# Autodesk Inventor assembly: Ensamble General
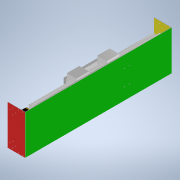
[picture p0: Inventor's stored thumbnail of the model, 180x180]
Saved by Autodesk Inventor 2021 (Build 250183000, 183)
## iProperties
Created: 2022-01-21
Part Number: Ensamble General
Document SubType Name: Assembly
Designer: deuts
Author: deuts
## Documents named in this file (11)
- C:\Users\deuts\Desktop\3dDesigne\SoladuraSemiAutomatizada\Ensamble General.iam
- C:\Users\deuts\Desktop\3dDesigne\SoladuraSemiAutomatizada\Soporte Tuerca.ipt
- C:\Users\deuts\Desktop\3dDesigne\SoladuraSemiAutomatizada\Tornillo 350.ipt
- C:\Users\deuts\Desktop\3dDesigne\SoladuraSemiAutomatizada\Tuerca 16.ipt
- C:\Users\deuts\Desktop\3dDesigne\SoladuraSemiAutomatizada\Acople Flexible.ipt
- C:\Users\deuts\Desktop\3dDesigne\SoladuraSemiAutomatizada\Motor Nema23.ipt
- C:\Users\deuts\Desktop\3dDesigne\SoladuraSemiAutomatizada\Rodamiento lineal.ipt
- C:\Users\deuts\Desktop\3dDesigne\SoladuraSemiAutomatizada\Soporte Motor.ipt
- C:\Users\deuts\Desktop\3dDesigne\SoladuraSemiAutomatizada\Riel.ipt
- C:\Users\deuts\Desktop\3dDesigne\SoladuraSemiAutomatizada\Caja - Base.ipt
- C:\Users\deuts\Desktop\3dDesigne\SoladuraSemiAutomatizada\CajaAux.ipt
## Components (14 placed, 10 different names)
1. Soporte Tuerca:1 — Mate:3, Mate:4, Mate:5, Angle:2, Angle:3, Mate:41, Flush:1, Mate:43, Flush:2
2. Tornillo 350:1 — Mate:3, Mate:6, Mate:7, Angle:1
3. Tuerca 16:1 — Mate:4, Mate:5, Angle:2
4. Acople Flexible:1 — Mate:6, Mate:7, Mate:8, Mate:9, Angle:1
5. Motor Nema23:1 — Mate:8, Mate:9, Angle:3, Mate:38, Angle:6, Mate:39, Flush:3, Flush:4
6. Soporte Motor:1 — Mate:38, Angle:6, Mate:39, Angle:7, Angle:8, Mate:46, Mate:47
7. Rodamiento lineal:1 — Mate:41, Flush:1, Mate:44, Mate:52
8. Rodamiento lineal:2 — Mate:43, Flush:2, Mate:45
9. Riel:1 — Mate:44, Angle:7, Flush:3, Mate:49, Mate:50
10. Riel:2 — Mate:45, Angle:8, Flush:4, Flush:5, Mate:48, Mate:51
11. Caja - Base:1 — Mate:46, Mate:47, Flush:5, Mate:50, Mate:51
12. Rodamiento lineal:3 — Mate:48
13. Rodamiento lineal:4 — Mate:49
14. CajaAux:1 — Mate:52
## Relationships (31: Mate 20, Angle 6, Flush 5)
- Mate:3: Soporte Tuerca:1 ↔ Tornillo 350:1
- Mate:4: Soporte Tuerca:1 ↔ Tuerca 16:1
- Mate:5: Soporte Tuerca:1 ↔ Tuerca 16:1
- Mate:6: Tornillo 350:1 ↔ Acople Flexible:1
- Mate:7 (-12 mm): Tornillo 350:1 ↔ Acople Flexible:1
- Mate:8: Acople Flexible:1 ↔ Motor Nema23:1
- Mate:9 (15 mm): Acople Flexible:1 ↔ Motor Nema23:1
- Angle:1 (0 deg): Tornillo 350:1 ↔ Acople Flexible:1
- Angle:2 (0 deg): Soporte Tuerca:1 ↔ Tuerca 16:1
- Angle:3 (0 deg): Soporte Tuerca:1 ↔ Motor Nema23:1
- Mate:38: Motor Nema23:1 ↔ Soporte Motor:1
- Angle:6 (0 deg): Motor Nema23:1 ↔ Soporte Motor:1
- Mate:39: Motor Nema23:1 ↔ Soporte Motor:1
- Mate:41 (7 mm): Soporte Tuerca:1 ↔ Rodamiento lineal:1
- Flush:1: Soporte Tuerca:1 ↔ Rodamiento lineal:1
- Mate:43 (7 mm): Soporte Tuerca:1 ↔ Rodamiento lineal:2
- Flush:2: Soporte Tuerca:1 ↔ Rodamiento lineal:2
- Mate:44: Rodamiento lineal:1 ↔ Riel:1
- Mate:45: Rodamiento lineal:2 ↔ Riel:2
- Angle:7 (0 deg): Soporte Motor:1 ↔ Riel:1
- Angle:8 (0 deg): Soporte Motor:1 ↔ Riel:2
- Flush:3 (41.7 mm): Motor Nema23:1 ↔ Riel:1
- Flush:4 (41.7 mm): Motor Nema23:1 ↔ Riel:2
- Mate:46: Soporte Motor:1 ↔ Caja - Base:1
- Mate:47: Soporte Motor:1 ↔ Caja - Base:1
- Flush:5 (0.5 mm): Riel:2 ↔ Caja - Base:1
- Mate:48: Riel:2 ↔ Rodamiento lineal:3
- Mate:49: Riel:1 ↔ Rodamiento lineal:4
- Mate:50: Riel:1 ↔ Caja - Base:1
- Mate:51: Riel:2 ↔ Caja - Base:1
- Mate:52: Rodamiento lineal:1 ↔ CajaAux:1
